# Autodesk Inventor assembly: Assey-N-N-body
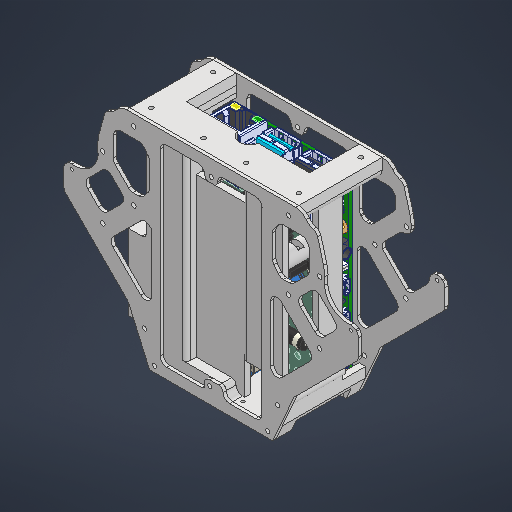
[picture p0: Inventor's stored thumbnail of the model, 512x512]
Saved by Autodesk Inventor 2026.1 (Build 301233020, 233B)
## iProperties
Created: 2026-03-17
Part Number: Assey-N-N-body
Document SubType Name: Assembly
Designer: kamada
Author: kamada
## Documents named in this file (6)
- D:\KiCad\KiProject\Nexus\Nexus-3dmodel\Assey-N-N-body.iam
- D:\KiCad\KiProject\Nexus\Nexus-3dmodel\NewBody-back.ipt
- D:\KiCad\KiProject\Nexus\Nexus-3dmodel\Nexus-pcb.iam
- D:\KiCad\KiProject\Nexus\Nexus-3dmodel\kosiss.ipt
- D:\KiCad\KiProject\Nexus\Nexus-3dmodel\N-NBody.ipt
- D:\KiCad\KiProject\Nexus\Nexus-3dmodel\NewBody.ipt
## Components (5 placed, 5 different names)
1. NewBody-back:1 — メイト:5, メイト:6, メイト:7, メイト:8, メイト:15, メイト:16, フラッシュ:3, フラッシュ:4, フラッシュ:5
2. Nexus-pcb:1 [sub-assembly] — メイト:1, メイト:2, メイト:3, メイト:4, メイト:15, メイト:16
3. kosiss:1
4. N-NBody:1 — フラッシュ:3, フラッシュ:4, フラッシュ:5, メイト:17, メイト:18, メイト:19
5. NewBody:1 — メイト:17, メイト:18, メイト:19
## Relationships (20: Mate 15, Flush 3, Symmetry 2)
- メイト:1 [Mate]: Nexus-pcb:1
- メイト:2 [Mate]: Nexus-pcb:1
- メイト:3 [Mate]: Nexus-pcb:1
- メイト:4 [Mate]: Nexus-pcb:1
- 対称度:1 [Symmetry]
- メイト:5 [Mate]: NewBody-back:1
- メイト:6 [Mate]: NewBody-back:1
- メイト:7 [Mate]: NewBody-back:1
- メイト:8 [Mate]: NewBody-back:1
- 対称度:2 [Symmetry]
- メイト:9 [Mate]
- メイト:14 [Mate]
- メイト:15 [Mate] (3 mm): NewBody-back:1 ↔ Nexus-pcb:1
- メイト:16 [Mate] (1 mm): NewBody-back:1 ↔ Nexus-pcb:1
- フラッシュ:3 [Flush]: NewBody-back:1 ↔ N-NBody:1
- フラッシュ:4 [Flush]: NewBody-back:1 ↔ N-NBody:1
- フラッシュ:5 [Flush]: NewBody-back:1 ↔ N-NBody:1
- メイト:17 [Mate]: N-NBody:1 ↔ NewBody:1
- メイト:18 [Mate]: N-NBody:1 ↔ NewBody:1
- メイト:19 [Mate]: N-NBody:1 ↔ NewBody:1
